# Autodesk Inventor assembly: BB25_block
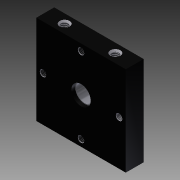
[picture p0: Inventor's stored thumbnail of the model, 180x180]
Saved by Autodesk Inventor 2012 (Build 160160000, 160)
## iProperties
Created: 2012-10-25
Part Number: BB25_block
Document SubType Name: Assembly
Designer: Andrew G. Meyer
Mass: 145.122 g
Surface Area: 156.104 cm^2
Volume: 46.2774 cm^3
Density: 3.13591 g/cm^3
Author: Andrew G. Meyer
## Documents named in this file (3)
- C:\Users\Andrew G. Meyer\Documents\Projects\BallBot\macro\CAD\BB25_block.iam
- C:\Users\Andrew G. Meyer\Documents\Projects\BallBot\macro\CAD\BB25_block.ipt
- C:\Users\Andrew G. Meyer\Documents\Projects\BallBot\macro\CAD\P80\br-8.ipt
## Components (2 placed, 2 different names)
1. BB25_block:1 — Insert:1
2. br-8:1 — Insert:1
## Relationships (1: Insert 1)
- Insert:1: BB25_block:1 ↔ br-8:1
